# Autodesk Inventor assembly: ヘッケンv2
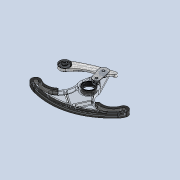
[picture p0: Inventor's stored thumbnail of the model, 180x180]
Saved by Autodesk Inventor 2020 (Build 240168000, 168)
## iProperties
Created: 2020-10-27
Part Number: ヘッケンv2
Document SubType Name: Assembly
Designer: AA19065
Author: AA19065
## Documents named in this file (9)
- C:\Users\happy\OneDrive\ドキュメント\賢一ファイル\SRDC\試作10-2\アセンブリ\ヘッケンv2.iam
- C:\Users\happy\OneDrive\ドキュメント\賢一ファイル\SRDC\試作10-2\脚クランク\揺動節.ipt
- C:\Users\happy\OneDrive\ドキュメント\賢一ファイル\SRDC\試作10-2\脚クランク\揺動節抑え.ipt
- C:\Users\happy\OneDrive\ドキュメント\賢一ファイル\SRDC\試作10-2\軸受け\オイレスw1.5f5-7n.ipt
- C:\Users\happy\OneDrive\ドキュメント\賢一ファイル\SRDC\試作10-2\軸受け\オイレスw5f6-10a.ipt
- C:\Users\happy\OneDrive\ドキュメント\賢一ファイル\SRDC\試作10-2\軸受け\オイレスw5f12-14n.ipt
- C:\Users\happy\OneDrive\ドキュメント\賢一ファイル\SRDC\試作10-2\ヘッケン\ヘッケンv2.ipt
- C:\Users\happy\OneDrive\ドキュメント\賢一ファイル\SRDC\試作10-2\ヘッケン\脚ゴム.ipt
- C:\Users\happy\OneDrive\ドキュメント\賢一ファイル\SRDC\試作10-2\ねじ\m3皿ネジ5 (1).ipt
## Components (9 placed, 8 different names)
1. 揺動節:1 — 挿入:8, 挿入:17
2. 揺動節抑え:1 — 挿入:12, 挿入:13
3. オイレスw1.5f5-7n:1 — 挿入:10, 挿入:17
4. オイレスw5f6-10a:1 — 挿入:8
5. オイレスw5f12-14n:1 — 挿入:11
6. ヘッケンv2:1 — 挿入:10, 挿入:11, 挿入:12, 挿入:13, 挿入:16, メイト:1, 挿入:18, 挿入:19
7. 脚ゴム:1 — 挿入:16, メイト:1
8. m3皿ネジ5 (1):1 — 挿入:19
9. m3皿ネジ5 (1):2 — 挿入:18
## Relationships (10: Insert 9, Mate 1)
- 挿入:8 [Insert]: 揺動節:1 ↔ オイレスw5f6-10a:1
- 挿入:10 [Insert]: オイレスw1.5f5-7n:1 ↔ ヘッケンv2:1
- 挿入:11 [Insert]: オイレスw5f12-14n:1 ↔ ヘッケンv2:1
- 挿入:12 [Insert]: 揺動節抑え:1 ↔ ヘッケンv2:1
- 挿入:13 [Insert]: 揺動節抑え:1 ↔ ヘッケンv2:1
- 挿入:16 [Insert]: ヘッケンv2:1 ↔ 脚ゴム:1
- メイト:1 [Mate] (-1.34 mm): ヘッケンv2:1 ↔ 脚ゴム:1
- 挿入:17 [Insert]: 揺動節:1 ↔ オイレスw1.5f5-7n:1
- 挿入:18 [Insert]: ヘッケンv2:1 ↔ m3皿ネジ5 (1):2
- 挿入:19 [Insert]: ヘッケンv2:1 ↔ m3皿ネジ5 (1):1
